# Autodesk Inventor assembly: hubble
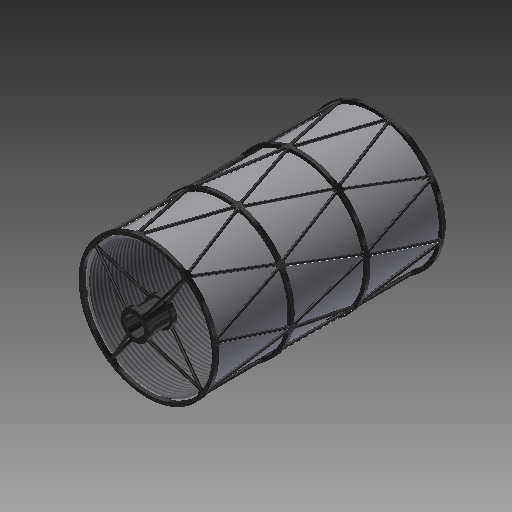
[picture p0: Inventor's stored thumbnail of the model, 512x512]
Saved by Autodesk Inventor 2018 (Build 220112000, 112)
## iProperties
Created: 2021-03-17
Part Number: hubble
Document SubType Name: Assembly
Designer: DELL
Author: DELL
## Documents named in this file (4)
- C:\Users\dell\Desktop\ES101 GROUP-13 PROJECT\FINAL MODEL\Resolved files\hubble.iam
- C:\Users\dell\Desktop\ES101 GROUP-13 PROJECT\INDIVIDUAL WORK\Dhruv\conical secondary baffle.ipt
- C:\Users\dell\Desktop\ES101 GROUP-13 PROJECT\INDIVIDUAL WORK\Dhruv\baffle.ipt
- C:\Users\dell\Desktop\ES101 GROUP-13 PROJECT\INDIVIDUAL WORK\Prey\metering truss.ipt
## Components (3 placed, 3 different names)
1. conical secondary baffle:1 — Mate:3, Mate:4
2. baffle:1 — Mate:1, Mate:2, Mate:3, Mate:4
3. metering truss:1 — Mate:1, Mate:2
## Relationships (4: Mate 4)
- Mate:1: baffle:1 ↔ metering truss:1
- Mate:2: baffle:1 ↔ metering truss:1
- Mate:3: conical secondary baffle:1 ↔ baffle:1
- Mate:4: conical secondary baffle:1 ↔ baffle:1
